# Autodesk Inventor assembly: СБ_Инфотабло
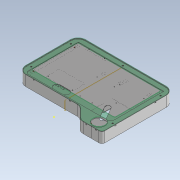
[picture p0: Inventor's stored thumbnail of the model, 180x180]
Saved by Autodesk Inventor 2021.2 (Build 252289000, 289)
## iProperties
Created: 2022-11-28
Part Number: СБ_Инфотабло
Document SubType Name: Assembly
Designer: Voodoo
Mass: 1296.68 g
Surface Area: 9308.33 cm^2
Volume: 1286.71 cm^3
Density: 1.00774 g/cm^3
Author: Voodoo
## Documents named in this file (15)
- C:\Users\Voodoo\Documents\Inventor\АБТ_Инфотабло\СБ_Инфотабло.iam
- C:\Users\Voodoo\Documents\Inventor\АБТ_Инфотабло\Блок питания LS-50-5_5V.ipt
- C:\Users\Voodoo\Documents\Inventor\АБТ_Инфотабло\Блок питания MA-60-12_12V.ipt
- C:\Users\Voodoo\Documents\Inventor\АБТ_Инфотабло\Медиа приставка GIBORIY X96 Mini 2.ipt
- C:\Users\Voodoo\Documents\Inventor\АБТ_Инфотабло\Скоба БП1.ipt
- C:\Users\Voodoo\Documents\Inventor\АБТ_Инфотабло\Скоба БП2.ipt
- C:\Users\Voodoo\Documents\Inventor\АБТ_Инфотабло\Кронштейн медиа приставки.ipt
- C:\Users\Voodoo\Documents\Inventor\АБТ_Инфотабло\Стекло.ipt
- C:\Users\Voodoo\Documents\Inventor\Content Center Files\R2021\ru-RU\AS 1427(05)\AS 1427 - M3 x 6(5) II.ipt
- C:\Users\Voodoo\Documents\Inventor\Content Center Files\R2021\ru-RU\ANSI B18.2.4.2M\ANSI B18.2.4.2M - M3x0,5 - 5,5.ipt
- C:\Users\Voodoo\Documents\Inventor\АБТ_Инфотабло\Плата контроллера.ipt
- C:\Users\Voodoo\Documents\Inventor\АБТ_Инфотабло\Матрица от ноутбука 15.6 NV156FHM-N42ipt.ipt
- C:\Users\Voodoo\Documents\Inventor\АБТ_Инфотабло\СБ_Короб задний.iam
- C:\Users\Voodoo\Documents\Inventor\АБТ_Инфотабло\СБ_Монтажный лист.iam
- C:\Users\Voodoo\Documents\Inventor\АБТ_Инфотабло\СБ_Корпус.iam
## Components (20 placed, 14 different names)
1. Матрица от ноутбука 15.6 NV156FHM-N42ipt:1
2. Медиа приставка GIBORIY X96 Mini 2:1 — Совмещение:56, Совмещение:57
3. Блок питания LS-50-5_5V:2 — Совмещение:68, Заподлицо:24, Совмещение:79, Заподлицо:25
4. Блок питания MA-60-12_12V:2 — Совмещение:61, Совмещение:68, Заподлицо:24, Заподлицо:26
5. Плата контроллера:1
6. Стекло:1
7. Скоба БП1:1 — Совмещение:61, Заподлицо:26
8. Скоба БП2:1 — Совмещение:79, Заподлицо:25
9. Кронштейн медиа приставки:2 — Совмещение:56, Совмещение:57
10. СБ_Короб задний:1 [sub-assembly]
11. СБ_Монтажный лист:1 [sub-assembly]
12. AS 1427 H - метрическая M3 x 6:1
13. AS 1427 H - метрическая M3 x 6:2
14. AS 1427 H - метрическая M3 x 6:3
15. AS 1427 H - метрическая M3 x 6:4
16. AS 1427 H - метрическая M3 x 6:5
17. ANSI B18.2.4.2M M3x0,5:1
18. ANSI B18.2.4.2M M3x0,5:3
19. ANSI B18.2.4.2M M3x0,5:4
20. СБ_Корпус:1 [sub-assembly]
## Relationships (44: Mate 24, Flush 11, Insert 8, Angle 1)
- [Flush]: СБ_Корпус:1
- [Flush]: СБ_Корпус:1
- [Flush]: СБ_Корпус:1
- [Flush]: СБ_Короб задний:1
- [Mate]: СБ_Монтажный лист:1 ↔ СБ_Корпус:1
- [Flush]: Матрица от ноутбука 15.6 NV156FHM-N42ipt:1 ↔ СБ_Корпус:1
- [Mate]: Скоба БП2:1 ↔ СБ_Монтажный лист:1
- [Mate]: Скоба БП1:1 ↔ СБ_Монтажный лист:1
- [Mate]: СБ_Короб задний:1 ↔ СБ_Монтажный лист:1
- [Mate] (5 mm): СБ_Короб задний:1 ↔ СБ_Корпус:1
- [Flush]: Стекло:1 ↔ СБ_Корпус:1
- [Flush]: Стекло:1 ↔ СБ_Корпус:1
- [Mate]: Стекло:1 ↔ СБ_Корпус:1
- [Insert] (2 mm): СБ_Монтажный лист:1 ↔ ANSI B18.2.4.2M M3x0,5:1
- [Insert]: AS 1427 H - метрическая M3 x 6:5 ↔ СБ_Корпус:1
- [Insert]: AS 1427 H - метрическая M3 x 6:3 ↔ СБ_Корпус:1
- [Insert]: AS 1427 H - метрическая M3 x 6:4 ↔ СБ_Корпус:1
- [Insert]: AS 1427 H - метрическая M3 x 6:1 ↔ СБ_Корпус:1
- [Insert]: AS 1427 H - метрическая M3 x 6:2 ↔ СБ_Корпус:1
- [Mate]: Медиа приставка GIBORIY X96 Mini 2:1 ↔ СБ_Монтажный лист:1
- Совмещение:56 [Mate] (1 mm): Медиа приставка GIBORIY X96 Mini 2:1 ↔ Кронштейн медиа приставки:2
- Совмещение:57 [Mate] (1 mm): Медиа приставка GIBORIY X96 Mini 2:1 ↔ Кронштейн медиа приставки:2
- [Mate]: Кронштейн медиа приставки:2 ↔ СБ_Монтажный лист:1
- Совмещение:61 [Mate]: Блок питания MA-60-12_12V:2 ↔ Скоба БП1:1
- [Mate]: Блок питания MA-60-12_12V:2 ↔ СБ_Монтажный лист:1
- [Mate]: Блок питания LS-50-5_5V:2 ↔ СБ_Монтажный лист:1
- Совмещение:68 [Mate] (20 mm): Блок питания LS-50-5_5V:2 ↔ Блок питания MA-60-12_12V:2
- [Mate] (52 mm): Блок питания LS-50-5_5V:2 ↔ СБ_Корпус:1
- [Mate]: Плата контроллера:1 ↔ СБ_Монтажный лист:1
- [Mate] (1.9 mm): Матрица от ноутбука 15.6 NV156FHM-N42ipt:1 ↔ СБ_Корпус:1
- [Mate] (1.7 mm): Матрица от ноутбука 15.6 NV156FHM-N42ipt:1 ↔ СБ_Корпус:1
- [Mate] (3 mm): СБ_Монтажный лист:1 ↔ СБ_Корпус:1
- [Mate] (3 mm): СБ_Монтажный лист:1 ↔ СБ_Корпус:1
- Заподлицо:24 [Flush]: Блок питания LS-50-5_5V:2 ↔ Блок питания MA-60-12_12V:2
- [Angle] (180 deg): Кронштейн медиа приставки:2 ↔ СБ_Корпус:1
- Совмещение:79 [Mate] (0.5 mm): Блок питания LS-50-5_5V:2 ↔ Скоба БП2:1
- Заподлицо:25 [Flush] (30 mm): Блок питания LS-50-5_5V:2 ↔ Скоба БП2:1
- Заподлицо:26 [Flush] (50 mm): Блок питания MA-60-12_12V:2 ↔ Скоба БП1:1
- [Flush]: Плата контроллера:1 ↔ СБ_Монтажный лист:1
- [Mate] (15 mm): Блок питания MA-60-12_12V:2 ↔ СБ_Корпус:1
- [Mate]: Плата контроллера:1 ↔ СБ_Монтажный лист:1
- [Insert] (2 mm): СБ_Монтажный лист:1 ↔ ANSI B18.2.4.2M M3x0,5:3
- [Insert] (2 mm): СБ_Монтажный лист:1 ↔ ANSI B18.2.4.2M M3x0,5:4
- [Mate]: Кронштейн медиа приставки:2 ↔ СБ_Монтажный лист:1
